# Autodesk Inventor assembly: artifact-assembly
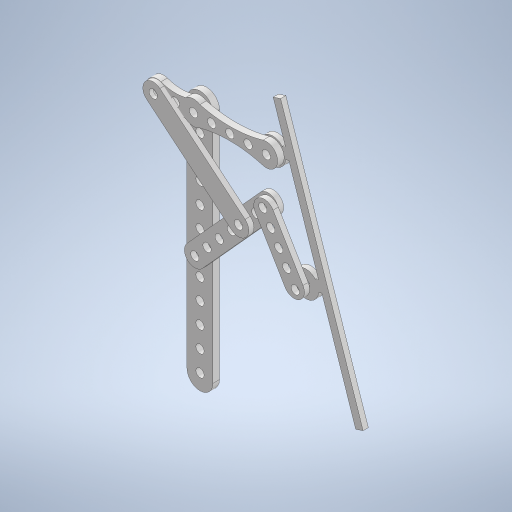
[picture p0: Inventor's stored thumbnail of the model, 512x512]
Saved by Autodesk Inventor 2024.1 (Build 281209000, 209)
## iProperties
Created: 2025-06-08
Part Number: artifact-assembly
Document SubType Name: Assembly
Designer: iwheard
Author: iwheard
## Documents named in this file (7)
- C:\Users\iwheard\Documents\0004-CAD\3D-cad-main\the-artifact\artifact-assembly.iam
- C:\Users\iwheard\Documents\0004-CAD\3D-cad-main\the-artifact\anchor-point.ipt
- C:\Users\iwheard\Documents\0004-CAD\3D-cad-main\see-saw-arm.ipt
- C:\Users\iwheard\Documents\0004-CAD\3D-cad-main\leaf-lid.ipt
- C:\Users\iwheard\Documents\0004-CAD\3D-cad-main\control-arm.ipt
- C:\Users\iwheard\Documents\0004-CAD\3D-cad-main\vertex-arm.ipt
- C:\Users\iwheard\Documents\0004-CAD\3D-cad-main\linkage-arm.ipt
## Components (6 placed, 6 different names)
1. anchor-point:1 — Flush:1, Flush:2, Flush:5
2. see-saw-arm:1 — Flush:1, Flush:2, Flush:3, Flush:4
3. leaf-lid:1 — Flush:3, Flush:4
4. control-arm:1 — Flush:5, Flush:6, Flush:7, Flush:8
5. vertex-arm:1 — Flush:6, Flush:7
6. linkage-arm:1 — Flush:8
## Relationships (8: Flush 8)
- Flush:1: anchor-point:1 ↔ see-saw-arm:1
- Flush:2: anchor-point:1 ↔ see-saw-arm:1
- Flush:3: see-saw-arm:1 ↔ leaf-lid:1
- Flush:4: see-saw-arm:1 ↔ leaf-lid:1
- Flush:5: anchor-point:1 ↔ control-arm:1
- Flush:6: control-arm:1 ↔ vertex-arm:1
- Flush:7: control-arm:1 ↔ vertex-arm:1
- Flush:8: control-arm:1 ↔ linkage-arm:1
